# Autodesk Inventor assembly: RT_ELE_003_350mmGutter.Harness1
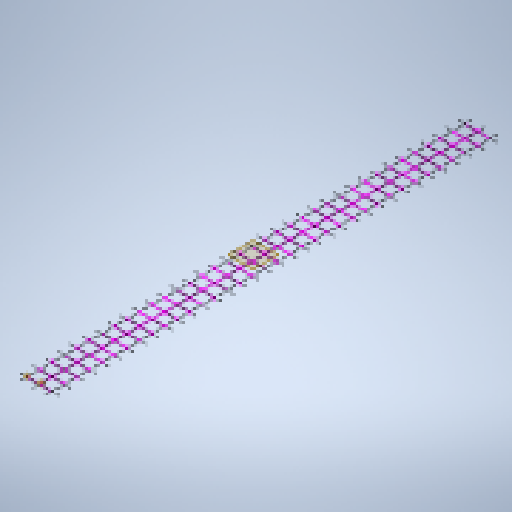
[picture p0: Inventor's stored thumbnail of the model, 512x512]
Saved by Autodesk Inventor 2025.3 (Build 293356000, 356)
## iProperties
Created: 2026-07-30
Part Number: RT_ELE_003_350mmGutter.Harness1
Document SubType Name: Assembly
Designer: louis
ParentFileIdentifier: 5|1|0|0|228|1|0|0|80|0|65|0|84|0|72|0|83|0|59|0|67|0|58|0|92|0|85|0|115|0|101|0|114|0|115|0|92|0|108|0|111|0|117|0|105|0|115|0|92|0|79|0|110|0|101|0|68|0|114|0|105|0|118|0|101|0|92|0|68|0|101|0|115|0|107|0|116|0|111|0|112|0|92|0|82|0|95|0|84|0|114|0|105|0|100|0|101|0|110|0|116|0|92|0|48|0|50|0|95|0|67|0|65|0|68|0|92|0|48|0|52|0|95|0|83|0|117|0|98|0|97|0|115|0|115|0|101|0|109|0|98|0|108|0|105|0|101|0|115|0|59|0|67|0|58|0|92|0|85|0|115|0|101|0|114|0|115|0|92|0|108|0|111|0|117|0|105|0|115|0|92|0|79|0|110|0|101|0|68|0|114|0|105|0|118|0|101|0|92|0|68|0|101|0|115|0|107|0|116|0|111|0|112|0|92|0|82|0|95|0|84|0|114|0|105|0|100|0|101|0|110|0|116|0|92|0|48|0|50|0|95|0|67|0|65|0|68|0|92|0|48|0|52|0|95|0|83|0|117|0|98|0|97|0|115|0|115|0|101|0|109|0|98|0|108|0|105|0|101|0|115|0|92|0|82|0|84|0|95|0|69|0|76|0|69|0|95|0|48|0|48|0|51|0|95|0|51|0|53|0|48|0|109|0|109|0|71|0|117|0|116|0|116|0|101|0|114|0|46|0|105|0|97|0|109|0|59|0|63|0|59|0|48|0|50|0|95|0|67|0|65|0|68|0|92|0|48|0|52|0|95|0|83|0|117|0|98|0|97|0|115|0|115|0|101|0|109|0|98|0|108|0|105|0|101|0|115|0|92|0|59|0|82|0|84|0|95|0|69|0|76|0|69|0|95|0|48|0|48|0|51|0|95|0|51|0|53|0|48|0|109|0|109|0|71|0|117|0|116|0|116|0|101|0|114|0|46|0|105|0|97|0|109|0|59|0|63|0|59|0|63|0|59|0|69|0|78|0|68|0|59|0|0|0|0|0|0|0|0|0|0|0|90|37|69|89|205|64|23|85|76|124|2|132|197|52|186|160|0|0|0|0|
HarnessSettings: <HarnessSettings><Defaults><Segments><Diameter value="0.200 in" fromwires="True"/><Offset value="0.100 in"/><ColorStyle value="Blue - Wall Paint - Glossy"/><RoundUp value=""/><BendRadius value="5" fromwires="False" ActiveCheck="False"/></Segments><Wires><GlobalSlack value="0.000000"/><RoundUp value=""/><PinEmbeddedLength value="1"/><PartEmbeddedLength value="1"/><SumOption value="0"/><InheritPointsOnDelSegment value="0"/><TangencyControlOnEndPoint value="1"/><NewTangencyControlOnEndPoint value="1"/></Wires><Splices><Offset value="0.100 in"/></Splices><RibbonCables><GlobalSlack value="0.0"/><Offset value="0.10 in"/></RibbonCables></Defaults><DisplayOptions><Segments><DisplayType value="Sweep"/></Segments><Wires><DisplayType value="Path"/><IsColorStyleFromLoom value="True"/></Wires><RibbonCables><DisplayType value="Sweep"/></RibbonCables></DisplayOptions><FileLocations><WireStyles><Location value="C:\Users\Public\Documents\Autodesk\Inventor 2025\Design Data\Cable &amp; Harness\en-US\Cable&amp;HarnessDefaultLibrary.iwl" UsingProjectDesignDataLocation="True"/><ModCode value="53e1dc8ebd40ef13fb5fbb200bc5ec51"/></WireStyles></FileLocations><NailboardSettings><DisplayOptions><Segments><DisplayType value="Sweep"/></Segments><Wires><DisplayType value="Path"/></Wires></DisplayOptions></NailboardSettings><ModelWithSurface value="True"/></HarnessSettings>
Author: louis
## Documents named in this file (2)
- C:\Users\louis\OneDrive\Desktop\R_Trident\02_CAD\04_Subassemblies\RT_ELE_003_350mmGutter\AIP\Cable and Harness\RT_ELE_003_350mmGutter.Harness1.iam
- C:\Users\louis\OneDrive\Desktop\R_Trident\02_CAD\04_Subassemblies\RT_ELE_003_350mmGutter\AIP\Cable and Harness\RT_ELE_003_350mmGutter.Harness1.ipt
## Components (1 placed, 1 different names)
1. Harness1
## Relationships (1: Flush 1)
- Flush:1 (-8 mm)
